# Autodesk Inventor assembly: outer
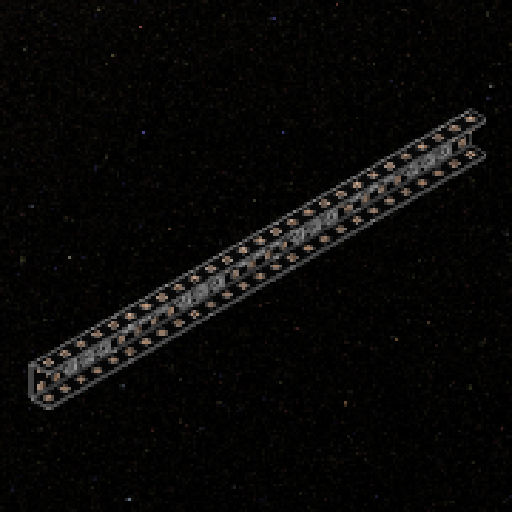
[picture p0: Inventor's stored thumbnail of the model, 512x512]
Saved by Autodesk Inventor 2024 (Build 280153000, 153)
## iProperties
Created: 2024-02-24
Part Number: outer
Document SubType Name: Assembly
Designer: Averey Ku
Author: Averey Ku
## Documents named in this file (8)
- D:\vex_robotics\hardware\cad\lil_zoom\chassis\drivebay\outer.iam
- D:\vex_robotics\hardware\cad\VEX-CAD-Inventor-1.41\Structure\C Channel\Aluminum 1x2x1\Alu C 1x2x1x27.ipt
- D:\vex_robotics\hardware\cad\VEX-CAD-Inventor-1.41\Motion\Shaft LS\Bearing Flat Low Profile.ipt
- D:\vex_robotics\hardware\cad\VEX-CAD-Inventor-1.41\Structure\Hardware\Nut Thin Nylock.ipt
- D:\vex_robotics\hardware\cad\VEX-CAD-Inventor-1.41\Motion\Spacers\Washer Steel\SWasher .375 OD x .062500.ipt
- D:\vex_robotics\hardware\cad\VEX-CAD-Inventor-1.41\Motion\Spacers\Washer Steel.ipt
- D:\vex_robotics\hardware\cad\VEX-CAD-Inventor-1.41\Structure\Hardware\Screw Steel - Star\SScrew Star Smooth 2.000.ipt
- D:\vex_robotics\hardware\cad\VEX-CAD-Inventor-1.41\Structure\Hardware\Screw Steel - Star.ipt
## Components (16 placed, 5 different names)
1. Alu C 1x2x1x27:1 — Insert:1, Mate:1, Insert:2, Mate:2, Insert:3, Mate:3, Insert:4, Mate:4, Insert:5, Mate:5, Insert:6, Mate:6, Insert:7, Mate:7, Insert:9, Insert:13, Insert:14, Insert:15
2. Bearing Flat Low Profile:1 — Insert:1, Mate:1
3. Bearing Flat Low Profile:2 — Insert:3, Mate:3
4. Bearing Flat Low Profile:3 — Insert:2, Mate:2, Insert:16
5. Bearing Flat Low Profile:4 — Insert:5, Mate:5
6. Bearing Flat Low Profile:5 — Insert:6, Mate:6, Insert:18
7. Bearing Flat Low Profile:6 — Insert:7, Mate:7
8. Bearing Flat Low Profile:7 — Insert:4, Mate:4, Insert:17
9. Nut Thin Nylock:1 — Insert:8, Insert:9
10. SWasher .375 OD x .062500:1 — Insert:8
11. Nut Thin Nylock:2 — Insert:13
12. Nut Thin Nylock:3 — Insert:14
13. Nut Thin Nylock:4 — Insert:15
14. SScrew Star Smooth 2.000:1 — Insert:16
15. SScrew Star Smooth 2.000:2 — Insert:17
16. SScrew Star Smooth 2.000:3 — Insert:18
## Relationships (22: Insert 15, Mate 7)
- Insert:1: Alu C 1x2x1x27:1 ↔ Bearing Flat Low Profile:1
- Mate:1: Alu C 1x2x1x27:1 ↔ Bearing Flat Low Profile:1
- Insert:2: Alu C 1x2x1x27:1 ↔ Bearing Flat Low Profile:3
- Mate:2: Alu C 1x2x1x27:1 ↔ Bearing Flat Low Profile:3
- Insert:3: Alu C 1x2x1x27:1 ↔ Bearing Flat Low Profile:2
- Mate:3: Alu C 1x2x1x27:1 ↔ Bearing Flat Low Profile:2
- Insert:4: Alu C 1x2x1x27:1 ↔ Bearing Flat Low Profile:7
- Mate:4: Alu C 1x2x1x27:1 ↔ Bearing Flat Low Profile:7
- Insert:5: Alu C 1x2x1x27:1 ↔ Bearing Flat Low Profile:4
- Mate:5: Alu C 1x2x1x27:1 ↔ Bearing Flat Low Profile:4
- Insert:6: Alu C 1x2x1x27:1 ↔ Bearing Flat Low Profile:5
- Mate:6: Alu C 1x2x1x27:1 ↔ Bearing Flat Low Profile:5
- Insert:7: Alu C 1x2x1x27:1 ↔ Bearing Flat Low Profile:6
- Mate:7: Alu C 1x2x1x27:1 ↔ Bearing Flat Low Profile:6
- Insert:8: Nut Thin Nylock:1 ↔ SWasher .375 OD x .062500:1
- Insert:9: Alu C 1x2x1x27:1 ↔ Nut Thin Nylock:1
- Insert:13: Alu C 1x2x1x27:1 ↔ Nut Thin Nylock:2
- Insert:14: Alu C 1x2x1x27:1 ↔ Nut Thin Nylock:3
- Insert:15: Alu C 1x2x1x27:1 ↔ Nut Thin Nylock:4
- Insert:16 (1.27 mm): Bearing Flat Low Profile:3 ↔ SScrew Star Smooth 2.000:1
- Insert:17 (1.27 mm): Bearing Flat Low Profile:7 ↔ SScrew Star Smooth 2.000:2
- Insert:18 (1.27 mm): Bearing Flat Low Profile:5 ↔ SScrew Star Smooth 2.000:3
